# Autodesk Inventor assembly: Case_principal
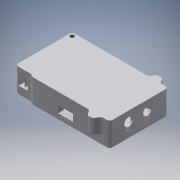
[picture p0: Inventor's stored thumbnail of the model, 180x180]
Saved by Autodesk Inventor 2019 (Build 230136000, 136)
## iProperties
Created: 2018-11-26
Part Number: Case_principal
Material: Generic
Document SubType Name: Assembly
Designer: cadcae
Author: cadcae
## Documents named in this file (11)
- D:\Hector\CAD_thesis\Case_principal.iam
- D:\Hector\CAD_thesis\Case2\Case_inferior_nuevo.ipt
- D:\Hector\CAD_thesis\PCB\tesis_schematic.iam
- D:\Hector\CAD_thesis\Inserts\94459A110_BRASS HEAT-SET INSERT FOR PLASTIC.ipt
- D:\Hector\CAD_thesis\Case_principal\Design Accelerator\Bolted Connection1.iam
- D:\Hector\CAD_thesis\Case2\Case_superior_nuevo.ipt
- D:\Hector\CAD_thesis\Inserts\94459A120_BRASS HEAT-SET INSERT FOR PLASTIC.ipt
- D:\Hector\CAD_thesis\Library\en-US\ISO 7046-1(1)\DIN EN ISO 7046-1 - M2 x 4 - 4.8 - H.ipt
- D:\Hector\CAD_thesis\Library\en-US\ISO 7046-1(1)\DIN EN ISO 7046-1 - M2 x 8 - 4.8 - H.ipt
- D:\Hector\CAD_thesis\LED\LED_3MM_ROJO.ipt
- D:\Hector\CAD_thesis\LED\LED_3MM_VERDE.ipt
## Components (15 placed, 10 different names)
1. Case_inferior_nuevo:1 — Flush:1, Flush:2, Flush:3, Mate:1, Mate:2, Mate:3, Mate:4, Mate:5, Mate:6, Flush:4, Flush:5, Flush:6, Angle:1, Angle:2, Angle:3, Flush:7, Mate:10, Angle:4, Mate:11, Mate:12, Flush:8, Mate:16, Mate:17
2. tesis_schematic:1 [sub-assembly] — Mate:1, Mate:2, Mate:3, Mate:7, Mate:9
3. 94459A110_BRASS HEAT-SET INSERT FOR PLASTIC:1 — Mate:4, Flush:6, Angle:1, Mate:8
4. 94459A110_BRASS HEAT-SET INSERT FOR PLASTIC:2 — Mate:5, Flush:5, Angle:2
5. 94459A110_BRASS HEAT-SET INSERT FOR PLASTIC:3 — Mate:6, Flush:4, Angle:3
6. Bolted Connection:1 [sub-assembly] — Mate:7, Mate:8, Mate:9
7. 94459A110_BRASS HEAT-SET INSERT FOR PLASTIC:4 — Flush:7, Mate:10, Angle:4
8. Case_superior_nuevo:1 — Mate:11, Mate:12, Flush:8, Flush:9, Flush:10, Mate:13, Mate:14, Angle:5, Angle:6, Mate:15, Mate:18, Mate:19, Mate:20, Mate:21, Angle:7, Angle:8
9. 94459A120_BRASS HEAT-SET INSERT FOR PLASTIC:1 — Flush:9, Mate:14, Angle:5
10. 94459A120_BRASS HEAT-SET INSERT FOR PLASTIC:2 — Flush:10, Mate:13, Angle:6
11. DIN EN ISO 7046-1 H M2 x 4 - 4.8 - H:1 — Mate:15
12. DIN EN ISO 7046-1 H M2 x 8 - 4.8 - H:1 — Mate:16
13. DIN EN ISO 7046-1 H M2 x 8 - 4.8 - H:2 — Mate:17
14. LED_3MM_ROJO:1 — Mate:19, Mate:21, Angle:8
15. LED_3MM_VERDE:1 — Mate:18, Mate:20, Angle:7
## Relationships (39: Mate 21, Flush 10, Angle 8)
- Flush:1: Case_inferior_nuevo:1
- Flush:2: Case_inferior_nuevo:1
- Flush:3: Case_inferior_nuevo:1
- Mate:1: Case_inferior_nuevo:1 ↔ tesis_schematic:1
- Mate:2 (0.5 mm): Case_inferior_nuevo:1 ↔ tesis_schematic:1
- Mate:3 (0.5 mm): Case_inferior_nuevo:1 ↔ tesis_schematic:1
- Mate:4: Case_inferior_nuevo:1 ↔ 94459A110_BRASS HEAT-SET INSERT FOR PLASTIC:1
- Mate:5: Case_inferior_nuevo:1 ↔ 94459A110_BRASS HEAT-SET INSERT FOR PLASTIC:2
- Mate:6: Case_inferior_nuevo:1 ↔ 94459A110_BRASS HEAT-SET INSERT FOR PLASTIC:3
- Flush:4: Case_inferior_nuevo:1 ↔ 94459A110_BRASS HEAT-SET INSERT FOR PLASTIC:3
- Flush:5: Case_inferior_nuevo:1 ↔ 94459A110_BRASS HEAT-SET INSERT FOR PLASTIC:2
- Flush:6: Case_inferior_nuevo:1 ↔ 94459A110_BRASS HEAT-SET INSERT FOR PLASTIC:1
- Angle:1 (0 deg): Case_inferior_nuevo:1 ↔ 94459A110_BRASS HEAT-SET INSERT FOR PLASTIC:1
- Angle:2 (0 deg): Case_inferior_nuevo:1 ↔ 94459A110_BRASS HEAT-SET INSERT FOR PLASTIC:2
- Angle:3 (0 deg): Case_inferior_nuevo:1 ↔ 94459A110_BRASS HEAT-SET INSERT FOR PLASTIC:3
- Mate:7: tesis_schematic:1 ↔ Bolted Connection:1
- Mate:8: 94459A110_BRASS HEAT-SET INSERT FOR PLASTIC:1 ↔ Bolted Connection:1
- Mate:9: tesis_schematic:1 ↔ Bolted Connection:1
- Flush:7: Case_inferior_nuevo:1 ↔ 94459A110_BRASS HEAT-SET INSERT FOR PLASTIC:4
- Mate:10: Case_inferior_nuevo:1 ↔ 94459A110_BRASS HEAT-SET INSERT FOR PLASTIC:4
- Angle:4 (0 deg): Case_inferior_nuevo:1 ↔ 94459A110_BRASS HEAT-SET INSERT FOR PLASTIC:4
- Mate:11: Case_inferior_nuevo:1 ↔ Case_superior_nuevo:1
- Mate:12: Case_inferior_nuevo:1 ↔ Case_superior_nuevo:1
- Flush:8: Case_inferior_nuevo:1 ↔ Case_superior_nuevo:1
- Flush:9: Case_superior_nuevo:1 ↔ 94459A120_BRASS HEAT-SET INSERT FOR PLASTIC:1
- Flush:10: Case_superior_nuevo:1 ↔ 94459A120_BRASS HEAT-SET INSERT FOR PLASTIC:2
- Mate:13: Case_superior_nuevo:1 ↔ 94459A120_BRASS HEAT-SET INSERT FOR PLASTIC:2
- Mate:14: Case_superior_nuevo:1 ↔ 94459A120_BRASS HEAT-SET INSERT FOR PLASTIC:1
- Angle:5 (0 deg): Case_superior_nuevo:1 ↔ 94459A120_BRASS HEAT-SET INSERT FOR PLASTIC:1
- Angle:6 (0 deg): Case_superior_nuevo:1 ↔ 94459A120_BRASS HEAT-SET INSERT FOR PLASTIC:2
- Mate:15: Case_superior_nuevo:1 ↔ DIN EN ISO 7046-1 H M2 x 4 - 4.8 - H:1
- Mate:16: Case_inferior_nuevo:1 ↔ DIN EN ISO 7046-1 H M2 x 8 - 4.8 - H:1
- Mate:17: Case_inferior_nuevo:1 ↔ DIN EN ISO 7046-1 H M2 x 8 - 4.8 - H:2
- Mate:18: Case_superior_nuevo:1 ↔ LED_3MM_VERDE:1
- Mate:19: Case_superior_nuevo:1 ↔ LED_3MM_ROJO:1
- Mate:20: Case_superior_nuevo:1 ↔ LED_3MM_VERDE:1
- Mate:21: Case_superior_nuevo:1 ↔ LED_3MM_ROJO:1
- Angle:7 (0 deg): Case_superior_nuevo:1 ↔ LED_3MM_VERDE:1
- Angle:8 (0 deg): Case_superior_nuevo:1 ↔ LED_3MM_ROJO:1
